# Autodesk Inventor assembly: Right Hook Whole Assembly_v2
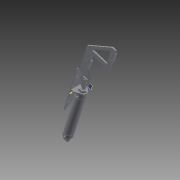
[picture p0: Inventor's stored thumbnail of the model, 180x180]
Saved by Autodesk Inventor 2013 (Build 170138000, 138)
## iProperties
Created: 2013-03-16
Part Number: Right Hook Whole Assembly_v2
Document SubType Name: Assembly
Designer: Arpan
Author: Arpan
## Documents named in this file (5)
- C:\Users\Arpan\Documents\GitHub\frc2013CAD\Midwest Climber\Right Hook Whole Assembly_v2.iam
- C:\Users\Arpan\Documents\GitHub\frc2013CAD\Midwest Climber\Right Hook Encoder Assembly.iam
- C:\Users\Arpan\Documents\GitHub\frc2013CAD\Midwest Climber\Piston Bracket Assembly.iam
- C:\Users\Arpan\Documents\GitHub\frc2013CAD\Midwest Climber\Ninja cylinder support bracket.ipt
- C:\Users\Arpan\Documents\GitHub\frc2013CAD\Midwest Climber\Limit Switch.ipt
## Components (4 placed, 4 different names)
1. Right Hook Encoder Assembly:1 [sub-assembly] — Mate:8, Mate:9, Mate:10, Mate:12, Mate:13, Angle:1
2. Piston Bracket Assembly:1 [sub-assembly] — Mate:4, Mate:5, Mate:6, Flush:1, Mate:8, Mate:9, Mate:10
3. Ninja cylinder support bracket:1 — Mate:4, Mate:5, Mate:6, Flush:1
4. Limit Switch:1 — Mate:12, Mate:13, Angle:1
## Relationships (10: Mate 8, Flush 1, Angle 1)
- Mate:4: Piston Bracket Assembly:1 ↔ Ninja cylinder support bracket:1
- Mate:5: Piston Bracket Assembly:1 ↔ Ninja cylinder support bracket:1
- Mate:6: Piston Bracket Assembly:1 ↔ Ninja cylinder support bracket:1
- Flush:1: Piston Bracket Assembly:1 ↔ Ninja cylinder support bracket:1
- Mate:8: Right Hook Encoder Assembly:1 ↔ Piston Bracket Assembly:1
- Mate:9: Right Hook Encoder Assembly:1 ↔ Piston Bracket Assembly:1
- Mate:10: Right Hook Encoder Assembly:1 ↔ Piston Bracket Assembly:1
- Mate:12: Right Hook Encoder Assembly:1 ↔ Limit Switch:1
- Mate:13: Right Hook Encoder Assembly:1 ↔ Limit Switch:1
- Angle:1 (0 deg): Right Hook Encoder Assembly:1 ↔ Limit Switch:1
